# Autodesk Inventor assembly: test_print
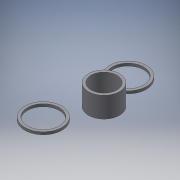
[picture p0: Inventor's stored thumbnail of the model, 180x180]
Saved by Autodesk Inventor 2019 (Build 230136000, 136)
## iProperties
Created: 2019-05-22
Part Number: test_print
Document SubType Name: Assembly
Designer: Nathan
Author: Nathan
## Documents named in this file (4)
- C:\Users\Nathan\workspace\fbd-brachium\cad\test_prints\test_print.iam
- C:\Users\Nathan\workspace\fbd-brachium\cad\test_prints\shaft.ipt
- C:\Users\Nathan\workspace\fbd-brachium\cad\test_prints\ring1.ipt
- C:\Users\Nathan\workspace\fbd-brachium\cad\test_prints\ring2.ipt
## Components (3 placed, 3 different names)
1. shaft:1 — Flush:1, Flush:2
2. ring1:1 — Flush:2
3. ring2:1 — Flush:1
## Relationships (2: Flush 2)
- Flush:1: shaft:1 ↔ ring2:1
- Flush:2: shaft:1 ↔ ring1:1
